# Autodesk Inventor assembly: RobotPallet
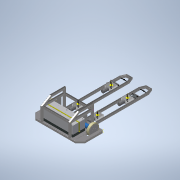
[picture p0: Inventor's stored thumbnail of the model, 180x180]
Saved by Autodesk Inventor 2022.1 (Build 261234000, 234)
## iProperties
Created: 2021-09-10
Part Number: RobotPallet
Material: Generic
Document SubType Name: Assembly
Designer: Andres
_SolveAssemblyDoc: Frame Generator Solve Assembly
_Version: 25.0.0
Author: Andres
## Documents named in this file (13)
- C:\Users\seb_0\Desktop\PDM\ProyectoRobotPallet\RobotPallet.iam
- C:\Users\seb_0\Desktop\PDM\ProyectoRobotPallet\Estructura Inferior\EstructuraInferior.iam
- C:\Users\seb_0\Desktop\PDM\ProyectoRobotPallet\Estructura Inferior\PlanchaBaseInferior.ipt
- C:\Users\seb_0\Desktop\PDM\ProyectoRobotPallet\Motor\BL Motor + Encoder + Gearbox + Rueda.iam
- C:\Users\seb_0\Desktop\PDM\ProyectoRobotPallet\SistemaDeElevacion\version2\SistemaElevacionV2.iam
- SistemaElevacion2.iam
- C:\Users\seb_0\Desktop\PDM\ProyectoRobotPallet\RuedasAuxiliares\Ruedas de soporte.iam
- C:\Users\seb_0\Desktop\PDM\ProyectoRobotPallet\Soportes\Rodamiento con soporte de pie\SKF_SYWK 30 YTH.iam
- C:\Users\seb_0\Desktop\PDM\ProyectoRobotPallet\RobotPallet\Frame\Frame_Superior.iam
- C:\Users\seb_0\Desktop\PDM\ProyectoRobotPallet\Componentes\Batería.ipt
- C:\Users\seb_0\Desktop\PDM\ProyectoRobotPallet\Soportes\Soporte_Gearbox.ipt
- C:\Users\seb_0\Desktop\PDM\ProyectoRobotPallet\Soportes\Soporte_Batería.ipt
- C:\Users\seb_0\Desktop\PDM\ProyectoRobotPallet\Soportes\Soporte_Batería2.ipt
## Components (21 placed, 11 different names)
1. EstructuraInferior:1 [sub-assembly] — Flush:1, Flush:13, Nivelación:23, Nivelación:24, Nivelación:25, Nivelación:26, Nivelación:27, Nivelación:28, Nivelación:29, Nivelación:30
2. PlanchaBaseInferior:1 — Flush:1, Coincidencia:28, Coincidencia:33, Coincidencia:34
3. BL Motor + Encoder + Gearbox + Rueda:1 [sub-assembly] — Mate:22, Coincidencia:23, Nivelación:15, Nivelación:25, Nivelación:26, Coincidencia:29, Coincidencia:30
4. BL Motor + Encoder + Gearbox + Rueda:2 [sub-assembly] — Mate:22, Nivelación:16, Coincidencia:24, Nivelación:27, Coincidencia:31, Coincidencia:32, Nivelación:28, Coincidencia:33
5. SistemaElevacion2:1 [sub-assembly] — Flush:11
6. SistemaElevacion2:2 [sub-assembly] — Flush:10, Flush:11
7. SistemaElevacion2:3 [sub-assembly] — Flush:10, Flush:12, Flush:13
8. SistemaElevacion2:4 [sub-assembly] — Flush:12
9. Ruedas de soporte:1 [sub-assembly] — Flush:14
10. Ruedas de soporte:2 [sub-assembly] — Flush:14
11. SKF_SYWK 30 YTH:1 [sub-assembly] — Nivelación:16, Coincidencia:24
12. SKF_SYWK 30 YTH:2 [sub-assembly] — Coincidencia:23, Nivelación:15
13. Frame_Superior:1 [sub-assembly]
14. Batería:1 — Coincidencia:25, Nivelación:19, Nivelación:22
15. Batería:2 — Coincidencia:25, Coincidencia:26, Nivelación:18, Nivelación:19, Nivelación:21, Nivelación:22, Coincidencia:28, Nivelación:23
16. Batería:3 — Coincidencia:26, Coincidencia:27, Nivelación:17, Nivelación:18, Nivelación:20, Nivelación:21
17. Batería:4 — Coincidencia:27, Nivelación:17, Nivelación:20, Nivelación:24
18. Soporte_Gearbox:1 — Coincidencia:29, Coincidencia:30
19. Soporte_Gearbox:2 — Coincidencia:31, Coincidencia:32
20. Soporte_Batería:1 — Coincidencia:34, Nivelación:29, Nivelación:30, Coincidencia:35, Coincidencia:36, Coincidencia:37
21. Soporte_Batería2:1 — Coincidencia:35, Coincidencia:36, Coincidencia:37
## Relationships (38: Flush 22, Mate 16)
- Flush:1: EstructuraInferior:1 ↔ PlanchaBaseInferior:1
- Mate:22: BL Motor + Encoder + Gearbox + Rueda:1 ↔ BL Motor + Encoder + Gearbox + Rueda:2
- Flush:10: SistemaElevacion2:2 ↔ SistemaElevacion2:3
- Flush:11: SistemaElevacion2:1 ↔ SistemaElevacion2:2
- Flush:12: SistemaElevacion2:3 ↔ SistemaElevacion2:4
- Flush:13: EstructuraInferior:1 ↔ SistemaElevacion2:3
- Flush:14: Ruedas de soporte:1 ↔ Ruedas de soporte:2
- Coincidencia:23 [Mate]: BL Motor + Encoder + Gearbox + Rueda:1 ↔ SKF_SYWK 30 YTH:2
- Nivelación:15 [Flush]: BL Motor + Encoder + Gearbox + Rueda:1 ↔ SKF_SYWK 30 YTH:2
- Nivelación:16 [Flush]: BL Motor + Encoder + Gearbox + Rueda:2 ↔ SKF_SYWK 30 YTH:1
- Coincidencia:24 [Mate]: BL Motor + Encoder + Gearbox + Rueda:2 ↔ SKF_SYWK 30 YTH:1
- Coincidencia:25 [Mate]: Batería:1 ↔ Batería:2
- Coincidencia:26 [Mate]: Batería:2 ↔ Batería:3
- Coincidencia:27 [Mate]: Batería:3 ↔ Batería:4
- Nivelación:17 [Flush]: Batería:3 ↔ Batería:4
- Nivelación:18 [Flush]: Batería:2 ↔ Batería:3
- Nivelación:19 [Flush]: Batería:1 ↔ Batería:2
- Nivelación:20 [Flush]: Batería:3 ↔ Batería:4
- Nivelación:21 [Flush]: Batería:2 ↔ Batería:3
- Nivelación:22 [Flush]: Batería:1 ↔ Batería:2
- Coincidencia:28 [Mate] (10 mm): PlanchaBaseInferior:1 ↔ Batería:2
- Nivelación:23 [Flush] (46 mm): EstructuraInferior:1 ↔ Batería:2
- Nivelación:24 [Flush] (202 mm): EstructuraInferior:1 ↔ Batería:4
- Nivelación:25 [Flush] (105 mm): EstructuraInferior:1 ↔ BL Motor + Encoder + Gearbox + Rueda:1
- Nivelación:26 [Flush] (70 mm): EstructuraInferior:1 ↔ BL Motor + Encoder + Gearbox + Rueda:1
- Nivelación:27 [Flush] (70 mm): EstructuraInferior:1 ↔ BL Motor + Encoder + Gearbox + Rueda:2
- Coincidencia:29 [Mate]: BL Motor + Encoder + Gearbox + Rueda:1 ↔ Soporte_Gearbox:1
- Coincidencia:30 [Mate]: BL Motor + Encoder + Gearbox + Rueda:1 ↔ Soporte_Gearbox:1
- Coincidencia:31 [Mate]: BL Motor + Encoder + Gearbox + Rueda:2 ↔ Soporte_Gearbox:2
- Coincidencia:32 [Mate]: BL Motor + Encoder + Gearbox + Rueda:2 ↔ Soporte_Gearbox:2
- Nivelación:28 [Flush] (105 mm): EstructuraInferior:1 ↔ BL Motor + Encoder + Gearbox + Rueda:2
- Coincidencia:33 [Mate]: PlanchaBaseInferior:1 ↔ BL Motor + Encoder + Gearbox + Rueda:2
- Coincidencia:34 [Mate]: PlanchaBaseInferior:1 ↔ Soporte_Batería:1
- Nivelación:29 [Flush] (201 mm): EstructuraInferior:1 ↔ Soporte_Batería:1
- Nivelación:30 [Flush] (45 mm): EstructuraInferior:1 ↔ Soporte_Batería:1
- Coincidencia:35 [Mate]: Soporte_Batería:1 ↔ Soporte_Batería2:1
- Coincidencia:36 [Mate]: Soporte_Batería:1 ↔ Soporte_Batería2:1
- Coincidencia:37 [Mate]: Soporte_Batería:1 ↔ Soporte_Batería2:1
